# Autodesk Inventor assembly: SoapAssemblyV2
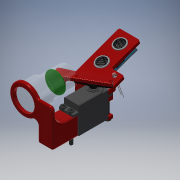
[picture p0: Inventor's stored thumbnail of the model, 180x180]
Saved by Autodesk Inventor 2018.3 (Build 223284000, 284)
## iProperties
Created: 2020-03-24
Part Number: SoapAssemblyV2
Document SubType Name: Assembly
Designer: Ivan
Author: Ivan
## Documents named in this file (13)
- C:\Users\Ivan\Documents\GitHub\Soap-dispenser\3D Model\SoapAssemblyV2.iam
- C:\Users\Ivan\Documents\GitHub\Soap-dispenser\3D Model\ServoSupport.ipt
- C:\Users\Ivan\Documents\GitHub\Soap-dispenser\3D Model\Servo MG995.ipt
- C:\Users\Ivan\Documents\GitHub\Soap-dispenser\3D Model\DispenserHead.ipt
- C:\Users\Ivan\Documents\GitHub\Soap-dispenser\3D Model\ServoArm2.ipt
- C:\Users\Ivan\Documents\GitHub\Soap-dispenser\3D Model\HC-SR04.ipt
- C:\Users\Ivan\Documents\GitHub\Soap-dispenser\3D Model\LED 5mm.ipt
- C:\Users\Ivan\Documents\GitHub\Soap-dispenser\3D Model\Arduino Pro Mini -Detailed -Blue.ipt
- C:\Users\Ivan\Documents\GitHub\Soap-dispenser\3D Model\ArmExtension.ipt
- C:\Users\Ivan\Documents\GitHub\Soap-dispenser\3D Model\MovingPlane.ipt
- C:\Users\Ivan\Documents\GitHub\Soap-dispenser\3D Model\UltrasonicBaseV2.ipt
- C:\Users\Ivan\Documents\GitHub\Soap-dispenser\3D Model\HexNut M4.ipt
- C:\Users\Ivan\Documents\Inventor\Content Center Files\R2018\en-US\ISO 10642(1)\ISO 10642 - M4 x  40.ipt
## Components (18 placed, 12 different names)
1. ServoSupport:1 — Mate:1, Flush:1, Mate:2, Mate:3, Mate:4, Mate:20, Mate:35, Mate:36, Mate:37, Mate:38, Mate:39, Mate:40
2. Servo MG995:1 — Mate:1, Flush:1, Mate:2, Insert:1, Angle:2, Mate:21, Mate:28, Flush:2, Insert:4, Insert:5
3. DispenserHead:1 — Mate:3, Mate:4
4. ServoArm2:1 — Insert:1, Mate:17, Mate:18, Mate:19
5. HC-SR04:1 — Mate:26, Angle:3, Mate:27
6. LED 5mm:1 — Mate:24, Mate:25
7. Arduino Pro Mini -Detailed -Blue:1 — Angle:2, Mate:47, Mate:48, Mate:49
8. ArmExtension:1 — Mate:17, Mate:18, Mate:19, Tangent:1
9. MovingPlane:1 — Tangent:1, Mate:20
10. UltrasonicBaseV2:1 — Mate:21, Mate:24, Mate:25, Mate:26, Angle:3, Mate:27, Mate:28, Flush:2, Mate:41, Mate:42, Mate:43, Mate:44, Mate:45, Mate:46, Mate:47, Mate:48, Mate:49, Mate:50, Insert:2, Insert:3
11. HexNut M4:1 — Mate:44, Mate:45, Mate:46
12. HexNut M4:2 — Mate:41, Mate:42, Mate:43
13. HexNut M4:3 — Mate:35, Mate:36, Mate:37
14. HexNut M4:4 — Mate:38, Mate:39, Mate:40
15. ISO 10642 M4 x  40:1 — Mate:50, Insert:2
16. ISO 10642 M4 x  40:2 — Insert:3
17. ISO 10642 M4 x  40:3 — Insert:4
18. ISO 10642 M4 x  40:4 — Insert:5
## Relationships (40: Mate 30, Insert 5, Flush 2, Angle 2, Tangent 1)
- Mate:1: ServoSupport:1 ↔ Servo MG995:1
- Flush:1: ServoSupport:1 ↔ Servo MG995:1
- Mate:2: ServoSupport:1 ↔ Servo MG995:1
- Mate:3: ServoSupport:1 ↔ DispenserHead:1
- Mate:4: ServoSupport:1 ↔ DispenserHead:1
- Insert:1: Servo MG995:1 ↔ ServoArm2:1
- Angle:2 (180 deg): Servo MG995:1 ↔ Arduino Pro Mini -Detailed -Blue:1
- Mate:17: ServoArm2:1 ↔ ArmExtension:1
- Mate:18: ServoArm2:1 ↔ ArmExtension:1
- Mate:19: ServoArm2:1 ↔ ArmExtension:1
- Tangent:1: ArmExtension:1 ↔ MovingPlane:1
- Mate:20: ServoSupport:1 ↔ MovingPlane:1
- Mate:21: Servo MG995:1 ↔ UltrasonicBaseV2:1
- Mate:24: LED 5mm:1 ↔ UltrasonicBaseV2:1
- Mate:25: LED 5mm:1 ↔ UltrasonicBaseV2:1
- Mate:26: HC-SR04:1 ↔ UltrasonicBaseV2:1
- Angle:3 (0 deg): HC-SR04:1 ↔ UltrasonicBaseV2:1
- Mate:27: HC-SR04:1 ↔ UltrasonicBaseV2:1
- Mate:28: Servo MG995:1 ↔ UltrasonicBaseV2:1
- Flush:2: Servo MG995:1 ↔ UltrasonicBaseV2:1
- Mate:35: ServoSupport:1 ↔ HexNut M4:3
- Mate:36: ServoSupport:1 ↔ HexNut M4:3
- Mate:37: ServoSupport:1 ↔ HexNut M4:3
- Mate:38: ServoSupport:1 ↔ HexNut M4:4
- Mate:39: ServoSupport:1 ↔ HexNut M4:4
- Mate:40: ServoSupport:1 ↔ HexNut M4:4
- Mate:41: UltrasonicBaseV2:1 ↔ HexNut M4:2
- Mate:42: UltrasonicBaseV2:1 ↔ HexNut M4:2
- Mate:43: UltrasonicBaseV2:1 ↔ HexNut M4:2
- Mate:44: UltrasonicBaseV2:1 ↔ HexNut M4:1
- Mate:45: UltrasonicBaseV2:1 ↔ HexNut M4:1
- Mate:46: UltrasonicBaseV2:1 ↔ HexNut M4:1
- Mate:47 (0.5 mm): Arduino Pro Mini -Detailed -Blue:1 ↔ UltrasonicBaseV2:1
- Mate:48 (1 mm): Arduino Pro Mini -Detailed -Blue:1 ↔ UltrasonicBaseV2:1
- Mate:49 (0.75 mm): Arduino Pro Mini -Detailed -Blue:1 ↔ UltrasonicBaseV2:1
- Mate:50: UltrasonicBaseV2:1 ↔ ISO 10642 M4 x  40:1
- Insert:2: UltrasonicBaseV2:1 ↔ ISO 10642 M4 x  40:1
- Insert:3: UltrasonicBaseV2:1 ↔ ISO 10642 M4 x  40:2
- Insert:4: Servo MG995:1 ↔ ISO 10642 M4 x  40:3
- Insert:5: Servo MG995:1 ↔ ISO 10642 M4 x  40:4
